# Autodesk Inventor assembly: mot_wheel
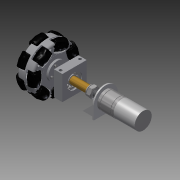
[picture p0: Inventor's stored thumbnail of the model, 180x180]
Saved by Autodesk Inventor 2015 (Build 190159000, 159)
## iProperties
Created: 2015-03-21
Part Number: mot_wheel
Document SubType Name: Assembly
Designer: Marcin
Author: Marcin
## Documents named in this file (9)
- C:\Users\Kuba\Dysk Google\synergia\Synergolf\model\GOLF\mot_wheel.iam
- C:\Users\Kuba\Dysk Google\synergia\Synergolf\model\GOLF\omni.iam
- C:\Users\Kuba\Dysk Google\synergia\Synergolf\model\GOLF\motor_all.iam
- C:\Users\Kuba\Dysk Google\synergia\Synergolf\model\GOLF\shaft.ipt
- C:\Users\Kuba\Dysk Google\synergia\Synergolf\model\GOLF\bearing_all.iam
- C:\Users\Kuba\Dysk Google\synergia\Synergolf\model\GOLF\Połączenie gwintowe1.iam
- C:\Users\Kuba\Dysk Google\synergia\Synergolf\model\GOLF\shaft_distance.ipt
- C:\Users\Kuba\Dysk Google\synergia\Synergolf\model\GOLF\DIN 988 - 8 x 14 x 1.ipt
- C:\Users\Kuba\Dysk Google\synergia\Synergolf\model\GOLF\DIN 555-5 - M8.ipt
## Components (8 placed, 8 different names)
1. omni:1 [sub-assembly] — Zestawiający:9, Zestawiający:10, Zestawiający:11, Zestawiający:12, Zestawiający:13
2. motor_all:1 [sub-assembly] — Równoległy:1, Równoległy:2, Równoległy:3, Zestawiający:5, Kąt:1, Zestawiający:8
3. shaft:1 — Zestawiający:5, Zestawiający:6, Zestawiający:7, Zestawiający:8, Zestawiający:9, Zestawiający:10, Zestawiający:11, Zestawiający:14, Zestawiający:17
4. bearing_all:1 [sub-assembly] — Zestawiający:6, Kąt:1, Zestawiający:7, Równoległy:4, Równoległy:5
5. Połączenie gwintowe:1 [sub-assembly] — Zestawiający:12, Zestawiający:13
6. shaft_distance:1 — Równoległy:4, Równoległy:5, Zestawiający:15
7. DIN 988 8 x 14 x 1:1 — Zestawiający:14, Zestawiający:15, Zestawiający:16
8. DIN 555 - zastąpiona przez DIN EN 24034 M8:1 — Zestawiający:16, Zestawiający:17
## Relationships (19: Mate 13, Flush 5, Angle 1)
- Równoległy:1 [Flush]: motor_all:1
- Równoległy:2 [Flush]: motor_all:1
- Równoległy:3 [Flush]: motor_all:1
- Zestawiający:5 [Mate] (2 mm): motor_all:1 ↔ shaft:1
- Zestawiający:6 [Mate]: shaft:1 ↔ bearing_all:1
- Kąt:1 [Angle] (0 deg): motor_all:1 ↔ bearing_all:1
- Zestawiający:7 [Mate]: shaft:1 ↔ bearing_all:1
- Zestawiający:8 [Mate]: motor_all:1 ↔ shaft:1
- Zestawiający:9 [Mate]: omni:1 ↔ shaft:1
- Zestawiający:10 [Mate]: omni:1 ↔ shaft:1
- Zestawiający:11 [Mate]: omni:1 ↔ shaft:1
- Zestawiający:12 [Mate]: omni:1 ↔ Połączenie gwintowe:1
- Zestawiający:13 [Mate]: omni:1 ↔ Połączenie gwintowe:1
- Równoległy:4 [Flush]: bearing_all:1 ↔ shaft_distance:1
- Równoległy:5 [Flush]: bearing_all:1 ↔ shaft_distance:1
- Zestawiający:14 [Mate]: shaft:1 ↔ DIN 988 8 x 14 x 1:1
- Zestawiający:15 [Mate]: shaft_distance:1 ↔ DIN 988 8 x 14 x 1:1
- Zestawiający:16 [Mate]: DIN 988 8 x 14 x 1:1 ↔ DIN 555 - zastąpiona przez DIN EN 24034 M8:1
- Zestawiający:17 [Mate]: shaft:1 ↔ DIN 555 - zastąpiona przez DIN EN 24034 M8:1
